# Autodesk Inventor assembly: TransmissionPulleyCenter
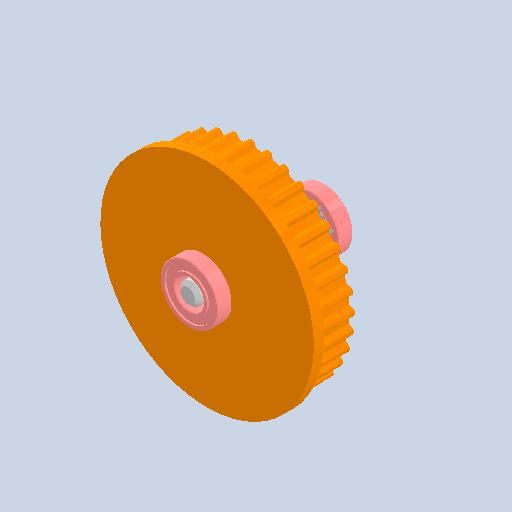
[picture p0: Inventor's stored thumbnail of the model, 512x512]
Saved by Autodesk Inventor 2022.2 (Build 262287030, 287C)
## iProperties
Created: 2022-01-08
Part Number: TransmissionPulleyCenter
Document SubType Name: Assembly
Designer: Jochen
Author: Jochen
## Documents named in this file (7)
- D:\Projects\Lisbeth\CAD\Common\Transmission\TransmissionPulleyCenter.iam
- D:\Projects\Lisbeth\CAD\Common\Transmission\TransmissionPulleyCentreAxis.ipt
- D:\Projects\Lisbeth\CAD\Common\Transmission\TransmissionCenterBigPulley.ipt
- D:\Projects\Lisbeth\CAD\Common\Bearing\bearing_8_4_2_sbn_MR84VA.ipt
- D:\Projects\Lisbeth\CAD\Common\Washer\Washer m2.5.ipt
- D:\Projects\Lisbeth\CAD\Common\Pulley\Pulley HTD 3M 10T.ipt
- Pulley HTD 3M 10T.ipt
## Components (7 placed, 5 different names)
1. MotorBeltTensionerAxis:1 — Mate:2, Mate:3, Mate:10, Mate:13, Mate:18, Mate:21, Mate:24
2. Center Pulley — Mate:21, Mate:22, Mate:23, Mate:25
3. bearing_8_4_2_sbn_MR84VA:1 — Mate:2, Mate:19
4. bearing_8_4_2_sbn_MR84VA:2 — Mate:3, Mate:12, Mate:18
5. Washer m2.5:1 — Mate:10, Mate:12, Mate:22
6. Washer m2.5:2 — Mate:13, Mate:19, Mate:23
7. Pulley HTD 3M 10T:1 — Mate:24, Mate:25
## Relationships (12: Mate 12)
- Mate:2: MotorBeltTensionerAxis:1 ↔ bearing_8_4_2_sbn_MR84VA:1
- Mate:3: MotorBeltTensionerAxis:1 ↔ bearing_8_4_2_sbn_MR84VA:2
- Mate:10: MotorBeltTensionerAxis:1 ↔ Washer m2.5:1
- Mate:12: bearing_8_4_2_sbn_MR84VA:2 ↔ Washer m2.5:1
- Mate:13: MotorBeltTensionerAxis:1 ↔ Washer m2.5:2
- Mate:18: MotorBeltTensionerAxis:1 ↔ bearing_8_4_2_sbn_MR84VA:2
- Mate:19: bearing_8_4_2_sbn_MR84VA:1 ↔ Washer m2.5:2
- Mate:21: MotorBeltTensionerAxis:1 ↔ Center Pulley
- Mate:22: Center Pulley ↔ Washer m2.5:1
- Mate:23: Center Pulley ↔ Washer m2.5:2
- Mate:24: MotorBeltTensionerAxis:1 ↔ Pulley HTD 3M 10T:1
- Mate:25: Center Pulley ↔ Pulley HTD 3M 10T:1
